# Autodesk Inventor assembly: WCP-0199
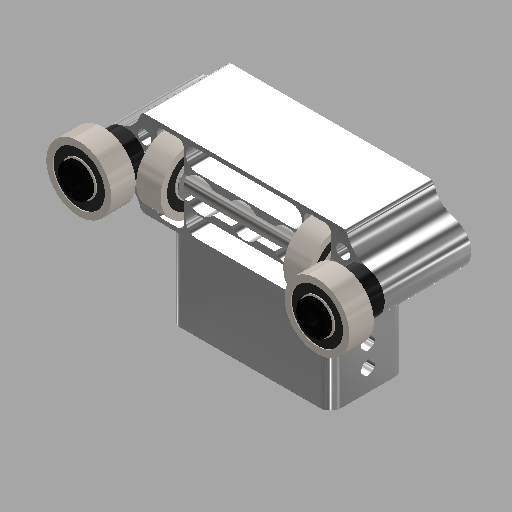
[picture p0: Inventor's stored thumbnail of the model, 512x512]
Saved by Autodesk Inventor 2024.3 (Build 283343000, 343)
## iProperties
Created: 2022-01-07
Part Number: WCP-0199
Description: STEP AP214
Document SubType Name: Assembly
Designer: Kenji
Mass: 165.023 g
Surface Area: 344.914 cm^2
Volume: 40.1768 cm^3
Density: 4.10741 g/cm^3
Sending System: SolidWorks 2020
Preprocessor: SwSTEP 2.0
Title: WCP-0199.step
Revision Number: ANY
## Documents named in this file (8)
- C:\Users\Kenji\Documents\GitHub\1622-2025-Reefscape-Offseason\COTS Library\Motion\Bearings\COTS_WCP-0199_InlineBearingBlock.iam
- C:\Users\Kenji\Documents\GitHub\1622-2025-Reefscape-Offseason\COTS Library\Motion\Bearings\WCP-0199\WCP-0199-001 Rev2.ipt
- C:\Users\Kenji\Documents\GitHub\1622-2025-Reefscape-Offseason\COTS Library\Motion\Bearings\WCP-0199\WCP-0199-004 Rev2.ipt
- C:\Users\Kenji\Documents\GitHub\1622-2025-Reefscape-Offseason\COTS Library\Motion\Bearings\WCP-0199\WCP-0199-003 Rev2_0.750 Bearing.ipt
- C:\Users\Kenji\Documents\GitHub\1622-2025-Reefscape-Offseason\COTS Library\Motion\Bearings\WCP-0199\WCP-0199-007 Rev2_0.750 Bearing.ipt
- C:\Users\Kenji\Documents\GitHub\1622-2025-Reefscape-Offseason\COTS Library\Motion\Bearings\WCP-0199\WCP-0474 Rev1.ipt
- C:\Users\Kenji\Documents\GitHub\1622-2025-Reefscape-Offseason\COTS Library\Motion\Bearings\WCP-0199\WCP-0212_0_250_radial_bearing.ipt
- C:\Users\Kenji\Documents\GitHub\1622-2025-Reefscape-Offseason\COTS Library\Motion\Bearings\WCP-0199\WCP-0039 Rev1.ipt
## Components (16 placed, 16 different names)
1. WCP-0199-001 Rev2_1 — Mate:2, Mate:3, Mate:6, Mate:7, Tangent:1, Tangent:2, Mate:13, Mate:14, Mate:21, Mate:22
2. WCP-0199-004 Rev2_2 — Mate:8, Tangent:1, Tangent:2, Mate:9, Mate:11, Tangent:3
3. WCP-0199-003 Rev2_0.750 Bearing_3 — Mate:25, Mate:26
4. WCP-0199-007 Rev2_0.750 Bearing_4 — Mate:13, Mate:14, Mate:15, Mate:16, Mate:17
5. WCP-0199-007 Rev2_0.750 Bearing_5 — Mate:19, Mate:20, Mate:22
6. WCP-0199-003 Rev2_0.750 Bearing_6 — Mate:27, Mate:28
7. WCP-0474 Rev1_7 — Mate:15, Mate:18, Mate:25, Mate:26
8. WCP-0474 Rev1_8 — Mate:23, Mate:24, Tangent:3, Mate:27, Mate:28
9. WCP-0212_0_250_radial_bearing_9 — Mate:16, Mate:17, Mate:18
10. WCP-0212_0_250_radial_bearing_10 — Mate:19, Mate:20, Mate:21, Mate:23, Mate:24
11. WCP-0212_0_250_radial_bearing_11 — Mate:11, Mate:12
12. WCP-0212_0_250_radial_bearing_12 — Mate:9, Mate:10
13. WCP-0039 Rev1_13 — Mate:4, Mate:5, Mate:7, Mate:8, Mate:12
14. WCP-0039 Rev1_14 — Mate:1, Mate:3, Mate:10
15. WCP-0039 Rev1_15 — Mate:4, Mate:6
16. WCP-0039 Rev1_16 — Mate:1, Mate:2, Mate:5
## Relationships (31: Mate 28, Tangent 3)
- Mate:1: WCP-0039 Rev1_14 ↔ WCP-0039 Rev1_16
- Mate:2: WCP-0199-001 Rev2_1 ↔ WCP-0039 Rev1_16
- Mate:3: WCP-0199-001 Rev2_1 ↔ WCP-0039 Rev1_14
- Mate:4: WCP-0039 Rev1_13 ↔ WCP-0039 Rev1_15
- Mate:5: WCP-0039 Rev1_13 ↔ WCP-0039 Rev1_16
- Mate:6: WCP-0199-001 Rev2_1 ↔ WCP-0039 Rev1_15
- Mate:7: WCP-0199-001 Rev2_1 ↔ WCP-0039 Rev1_13
- Mate:8: WCP-0199-004 Rev2_2 ↔ WCP-0039 Rev1_13
- Tangent:1: WCP-0199-001 Rev2_1 ↔ WCP-0199-004 Rev2_2
- Tangent:2: WCP-0199-001 Rev2_1 ↔ WCP-0199-004 Rev2_2
- Mate:9: WCP-0199-004 Rev2_2 ↔ WCP-0212_0_250_radial_bearing_12
- Mate:10: WCP-0212_0_250_radial_bearing_12 ↔ WCP-0039 Rev1_14
- Mate:11: WCP-0199-004 Rev2_2 ↔ WCP-0212_0_250_radial_bearing_11
- Mate:12: WCP-0212_0_250_radial_bearing_11 ↔ WCP-0039 Rev1_13
- Mate:13: WCP-0199-001 Rev2_1 ↔ WCP-0199-007 Rev2_0.750 Bearing_4
- Mate:14: WCP-0199-001 Rev2_1 ↔ WCP-0199-007 Rev2_0.750 Bearing_4
- Mate:15: WCP-0199-007 Rev2_0.750 Bearing_4 ↔ WCP-0474 Rev1_7
- Mate:16: WCP-0199-007 Rev2_0.750 Bearing_4 ↔ WCP-0212_0_250_radial_bearing_9
- Mate:17: WCP-0199-007 Rev2_0.750 Bearing_4 ↔ WCP-0212_0_250_radial_bearing_9
- Mate:18: WCP-0474 Rev1_7 ↔ WCP-0212_0_250_radial_bearing_9
- Mate:19: WCP-0199-007 Rev2_0.750 Bearing_5 ↔ WCP-0212_0_250_radial_bearing_10
- Mate:20: WCP-0199-007 Rev2_0.750 Bearing_5 ↔ WCP-0212_0_250_radial_bearing_10
- Mate:21: WCP-0199-001 Rev2_1 ↔ WCP-0212_0_250_radial_bearing_10
- Mate:22: WCP-0199-001 Rev2_1 ↔ WCP-0199-007 Rev2_0.750 Bearing_5
- Mate:23: WCP-0474 Rev1_8 ↔ WCP-0212_0_250_radial_bearing_10
- Mate:24: WCP-0474 Rev1_8 ↔ WCP-0212_0_250_radial_bearing_10
- Tangent:3: WCP-0199-004 Rev2_2 ↔ WCP-0474 Rev1_8
- Mate:25: WCP-0199-003 Rev2_0.750 Bearing_3 ↔ WCP-0474 Rev1_7
- Mate:26: WCP-0199-003 Rev2_0.750 Bearing_3 ↔ WCP-0474 Rev1_7
- Mate:27: WCP-0199-003 Rev2_0.750 Bearing_6 ↔ WCP-0474 Rev1_8
- Mate:28: WCP-0199-003 Rev2_0.750 Bearing_6 ↔ WCP-0474 Rev1_8
